# Autodesk Inventor assembly: probe-port-mesh-welded
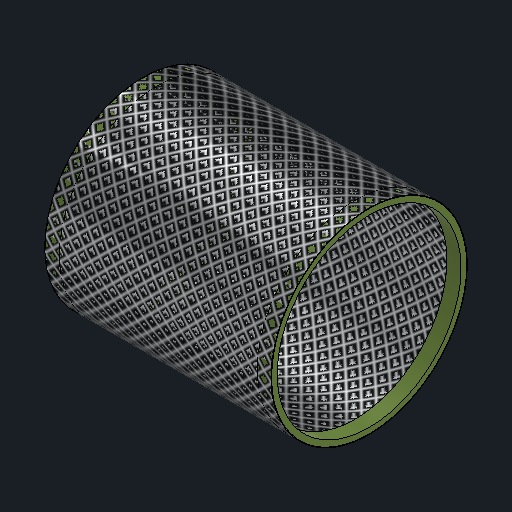
[picture p0: Inventor's stored thumbnail of the model, 512x512]
Saved by Autodesk Inventor 2026 (Build 300175050, 175E)
## iProperties
Created: 2024-06-28
Part Number: probe-port-mesh-welded
Document SubType Name: Assembly
Designer: kuzmin
Author: kuzmin
## Documents named in this file (3)
- C:\Users\queez\Dropbox\Drawings\PIHTI\Plasma Vessel\probe-port-mesh-welded.iam
- C:\Users\queez\Dropbox\Drawings\PIHTI\Plasma Vessel\flange-mesh-ring.ipt
- C:\Users\queez\Dropbox\Drawings\PIHTI\Plasma Vessel\probe-port-mesh.ipt
## Components (3 placed, 2 different names)
1. flange-mesh-ring:1 — Rigid:2
2. flange-mesh-ring:2
3. probe-port-mesh:1 — Rigid:2
## Relationships (3: WeldJoint 2, Mate 1)
- [Mate]: flange-mesh-ring:1 ↔ flange-mesh-ring:2
- [WeldJoint]: flange-mesh-ring:2 ↔ probe-port-mesh:1
- Rigid:2 [WeldJoint]: flange-mesh-ring:1 ↔ probe-port-mesh:1
